# Autodesk Inventor assembly: Reflow Oven
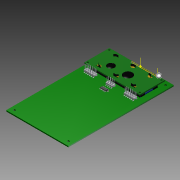
[picture p0: Inventor's stored thumbnail of the model, 180x180]
Saved by Autodesk Inventor 2015 (Build 190159000, 159)
## iProperties
Created: 2014-07-30
Part Number: Reflow Oven
Document SubType Name: Assembly
Designer: simon
Author: simon
## Documents named in this file (3)
- D:\Develop\Reflow Oven USB\Inventor\Reflow Oven.iam
- D:\Develop\Reflow Oven USB\Inventor\Reflow Front.iam
- D:\Develop\Reflow Oven USB\Inventor\LCD 16x2 Module.iam
## Components (2 placed, 2 different names)
1. Reflow Front:1 [sub-assembly] — Mate:1, Flush:1, Mate:2
2. LCD 16x2 Module:1 [sub-assembly] — Mate:1, Flush:1, Mate:2
## Relationships (3: Mate 2, Flush 1)
- Mate:1: Reflow Front:1 ↔ LCD 16x2 Module:1
- Flush:1: Reflow Front:1 ↔ LCD 16x2 Module:1
- Mate:2: Reflow Front:1 ↔ LCD 16x2 Module:1
